# Autodesk Inventor assembly: Assembly
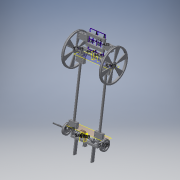
[picture p0: Inventor's stored thumbnail of the model, 180x180]
Saved by Autodesk Inventor 2018 (Build 220112000, 112)
## iProperties
Created: 2017-11-06
Part Number: Assembly
Document SubType Name: Assembly
Designer: David Cutting
Author: David Cutting
## Documents named in this file (17)
- C:\Users\Prakash\Documents\Inventor\MousetrapGit\Assembly.iam
- C:\Users\Prakash\Documents\Inventor\MousetrapGit\frontChassis_final.ipt
- C:\Users\Prakash\Documents\Inventor\MousetrapGit\carbonFiberTube.ipt
- C:\Users\Prakash\Documents\Inventor\MousetrapGit\clampCap.ipt
- C:\Users\Prakash\Documents\Inventor\MousetrapGit\rearChassis_final.ipt
- C:\Users\Prakash\Documents\Inventor\MousetrapGit\mousetrapHolder.ipt
- C:\Users\Prakash\Documents\Inventor\MousetrapGit\535018\bearings.ipt
- C:\Users\Prakash\Documents\Inventor\MousetrapGit\98873A200_MOISTURE-RESISTANT ACETAL THREADED ROD.ipt
- C:\Users\Prakash\Documents\Inventor\MousetrapGit\nutSecurer.ipt
- C:\Users\Prakash\Documents\Inventor\MousetrapGit\99223A029_ACETAL HEX NUT.ipt
- C:\Users\Prakash\Documents\Inventor\MousetrapGit\wheel.ipt
- C:\Users\Prakash\Documents\Inventor\MousetrapGit\spindleRod.ipt
- C:\Users\Prakash\Documents\Inventor\MousetrapGit\wheelSpindle.ipt
- C:\Users\Prakash\Documents\Inventor\MousetrapGit\intermediateSpindle.ipt
- C:\Users\Prakash\Documents\Inventor\MousetrapGit\wingnut_final.ipt
- C:\Users\Prakash\Documents\Inventor\MousetrapGit\washeript.ipt
- C:\Users\Prakash\Documents\Inventor\MousetrapGit\smallWheel.ipt
## Components (50 placed, 16 different names)
1. frontChassis_final:1 — Mate:1, Mate:2, Mate:3, Mate:4, Angle:3, Flush:3, Angle:4, Flush:4, Mate:16, Mate:17, Mate:18, Mate:19, Mate:24, Mate:25, Mate:26, Mate:27, Mate:52, Angle:8
2. carbonFiberTube:1 — Mate:1, Mate:2, Mate:6, Mate:9, Mate:10, Mate:12, Mate:14
3. carbonFiberTube:2 — Mate:3, Mate:4, Mate:5, Mate:7, Mate:8, Mate:11, Mate:13, Mate:15
4. clampCap:1 — Mate:8, Angle:1, Flush:1
5. clampCap:2 — Mate:9, Angle:2, Flush:2
6. rearChassis_final:1 — Mate:5, Mate:6, Mate:7, Angle:1, Flush:1, Angle:2, Flush:2, Mate:20, Mate:21, Mate:22, Mate:23, Mate:31, Angle:7
7. clampCap:3 — Mate:10, Angle:3, Flush:3
8. clampCap:4 — Mate:11, Angle:4, Flush:4
9. mousetrapHolder:1 — Mate:12, Mate:13, Angle:5, Flush:5, Angle:6, Flush:6
10. clampCap:5 — Mate:15, Angle:6, Flush:6
11. clampCap:6 — Mate:14, Angle:5, Flush:5
12. bearings:1 — Mate:16, Mate:17, Mate:29, Mate:35
13. bearings:2 — Mate:26, Mate:27
14. bearings:3 — Mate:18, Mate:19, Mate:28, Mate:39
15. bearings:4 — Mate:20, Mate:21, Mate:33
16. bearings:5 — Mate:24, Mate:25
17. bearings:6 — Mate:22, Mate:23, Mate:30, Mate:37
18. 98873A200_MOISTURE-RESISTANT ACETAL THREADED ROD:1 — Mate:30, Mate:31, Mate:32, Mate:36, Mate:40, Mate:42, Mate:49, Mate:50, Mate:62, Mate:64, Mate:65, Mate:76, Mate:79, Mate:80, Mate:82, Flush:7
19. 98873A200_MOISTURE-RESISTANT ACETAL THREADED ROD:2 — Mate:28, Mate:29, Mate:34, Mate:38, Mate:44, Mate:46, Mate:53, Mate:63, Mate:66, Mate:67, Mate:77, Mate:81, Mate:83, Mate:84, Flush:8, Mate:93, Mate:96
20. nutSecurer:1 — Mate:34, Mate:35, Mate:47
21. nutSecurer:2 — Mate:36, Mate:37, Mate:41
22. nutSecurer:3 — Mate:32, Mate:33, Mate:43
23. nutSecurer:4 — Mate:38, Mate:39, Mate:45
24. 99223A029_ACETAL HEX NUT:1 — Mate:40, Mate:41, Mate:68
25. 99223A029_ACETAL HEX NUT:2 — Mate:42, Mate:43, Mate:69
26. 99223A029_ACETAL HEX NUT:3 — Mate:46, Mate:47, Mate:70
27. 99223A029_ACETAL HEX NUT:4 — Mate:44, Mate:45, Mate:71
28. wheel:2 — Mate:50, Angle:11, Mate:74, Mate:87
29. wheel:4 — Mate:49, Angle:12, Mate:75, Mate:88
30. spindleRod:1 — Mate:52, Mate:54
31. wheelSpindle:1 — Mate:53, Flush:9
32. intermediateSpindle:1 — Mate:54, Flush:9
33. wingnut_final:1 — Mate:55, Mate:56, Mate:57, Mate:62, Angle:7
34. wingnut_final:2 — Mate:58, Mate:59, Mate:60, Mate:61, Mate:63, Angle:8
35. 99223A029_ACETAL HEX NUT:5 — Mate:55, Mate:56, Mate:57
36. 99223A029_ACETAL HEX NUT:6 — Mate:58, Mate:59, Mate:60, Mate:61
37. 99223A029_ACETAL HEX NUT:7 — Mate:64, Mate:68, Angle:12, Mate:75
38. 99223A029_ACETAL HEX NUT:8 — Mate:65, Mate:69, Angle:11, Mate:74
39. 99223A029_ACETAL HEX NUT:9 — Mate:67, Mate:71, Angle:14, Mate:97
40. 99223A029_ACETAL HEX NUT:10 — Mate:66, Mate:70, Angle:13, Mate:94
41. 99223A029_ACETAL HEX NUT:11 — Mate:77, Mate:91, Flush:8
42. 99223A029_ACETAL HEX NUT:12 — Mate:76, Mate:89
43. 99223A029_ACETAL HEX NUT:13 — Mate:79, Mate:90, Flush:7
44. washeript:1 — Mate:82, Mate:87, Mate:90
45. washeript:2 — Mate:81, Mate:91, Mate:98
46. washeript:4 — Mate:80, Mate:88, Mate:89
47. washeript:5 — Mate:83, Mate:92, Mate:95
48. 99223A029_ACETAL HEX NUT:14 — Mate:84, Mate:92
49. smallWheel:1 — Mate:93, Angle:13, Mate:94, Mate:95
50. smallWheel:2 — Mate:96, Angle:14, Mate:97, Mate:98
## Relationships (112: Mate 91, Angle 12, Flush 9)
- Mate:1: frontChassis_final:1 ↔ carbonFiberTube:1
- Mate:2: frontChassis_final:1 ↔ carbonFiberTube:1
- Mate:3: frontChassis_final:1 ↔ carbonFiberTube:2
- Mate:4: frontChassis_final:1 ↔ carbonFiberTube:2
- Mate:5: carbonFiberTube:2 ↔ rearChassis_final:1
- Mate:6: carbonFiberTube:1 ↔ rearChassis_final:1
- Mate:7: carbonFiberTube:2 ↔ rearChassis_final:1
- Mate:8: carbonFiberTube:2 ↔ clampCap:1
- Angle:1 (0 deg): clampCap:1 ↔ rearChassis_final:1
- Flush:1: clampCap:1 ↔ rearChassis_final:1
- Mate:9: carbonFiberTube:1 ↔ clampCap:2
- Angle:2 (0 deg): clampCap:2 ↔ rearChassis_final:1
- Flush:2: clampCap:2 ↔ rearChassis_final:1
- Mate:10: carbonFiberTube:1 ↔ clampCap:3
- Angle:3 (0 deg): frontChassis_final:1 ↔ clampCap:3
- Flush:3: frontChassis_final:1 ↔ clampCap:3
- Mate:11: carbonFiberTube:2 ↔ clampCap:4
- Angle:4 (0 deg): frontChassis_final:1 ↔ clampCap:4
- Flush:4: frontChassis_final:1 ↔ clampCap:4
- Mate:12: carbonFiberTube:1 ↔ mousetrapHolder:1
- Mate:13: carbonFiberTube:2 ↔ mousetrapHolder:1
- Mate:14: carbonFiberTube:1 ↔ clampCap:6
- Angle:5 (0 deg): mousetrapHolder:1 ↔ clampCap:6
- Flush:5: mousetrapHolder:1 ↔ clampCap:6
- Mate:15: carbonFiberTube:2 ↔ clampCap:5
- Angle:6 (0 deg): mousetrapHolder:1 ↔ clampCap:5
- Flush:6: mousetrapHolder:1 ↔ clampCap:5
- Mate:16: frontChassis_final:1 ↔ bearings:1
- Mate:17: frontChassis_final:1 ↔ bearings:1
- Mate:18: frontChassis_final:1 ↔ bearings:3
- Mate:19: frontChassis_final:1 ↔ bearings:3
- Mate:20: rearChassis_final:1 ↔ bearings:4
- Mate:21: rearChassis_final:1 ↔ bearings:4
- Mate:22: rearChassis_final:1 ↔ bearings:6
- Mate:23: rearChassis_final:1 ↔ bearings:6
- Mate:24: frontChassis_final:1 ↔ bearings:5
- Mate:25: frontChassis_final:1 ↔ bearings:5
- Mate:26: frontChassis_final:1 ↔ bearings:2
- Mate:27: frontChassis_final:1 ↔ bearings:2
- Mate:28: bearings:3 ↔ 98873A200_MOISTURE-RESISTANT ACETAL THREADED ROD:2
- Mate:29: bearings:1 ↔ 98873A200_MOISTURE-RESISTANT ACETAL THREADED ROD:2
- Mate:30: bearings:6 ↔ 98873A200_MOISTURE-RESISTANT ACETAL THREADED ROD:1
- Mate:31: rearChassis_final:1 ↔ 98873A200_MOISTURE-RESISTANT ACETAL THREADED ROD:1
- Mate:32: 98873A200_MOISTURE-RESISTANT ACETAL THREADED ROD:1 ↔ nutSecurer:3
- Mate:33: bearings:4 ↔ nutSecurer:3
- Mate:34: 98873A200_MOISTURE-RESISTANT ACETAL THREADED ROD:2 ↔ nutSecurer:1
- Mate:35: bearings:1 ↔ nutSecurer:1
- Mate:36: 98873A200_MOISTURE-RESISTANT ACETAL THREADED ROD:1 ↔ nutSecurer:2
- Mate:37: bearings:6 ↔ nutSecurer:2
- Mate:38: 98873A200_MOISTURE-RESISTANT ACETAL THREADED ROD:2 ↔ nutSecurer:4
- Mate:39: bearings:3 ↔ nutSecurer:4
- Mate:40: 98873A200_MOISTURE-RESISTANT ACETAL THREADED ROD:1 ↔ 99223A029_ACETAL HEX NUT:1
- Mate:41: nutSecurer:2 ↔ 99223A029_ACETAL HEX NUT:1
- Mate:42: 98873A200_MOISTURE-RESISTANT ACETAL THREADED ROD:1 ↔ 99223A029_ACETAL HEX NUT:2
- Mate:43: nutSecurer:3 ↔ 99223A029_ACETAL HEX NUT:2
- Mate:44: 98873A200_MOISTURE-RESISTANT ACETAL THREADED ROD:2 ↔ 99223A029_ACETAL HEX NUT:4
- Mate:45: nutSecurer:4 ↔ 99223A029_ACETAL HEX NUT:4
- Mate:46: 98873A200_MOISTURE-RESISTANT ACETAL THREADED ROD:2 ↔ 99223A029_ACETAL HEX NUT:3
- Mate:47: nutSecurer:1 ↔ 99223A029_ACETAL HEX NUT:3
- Mate:49: 98873A200_MOISTURE-RESISTANT ACETAL THREADED ROD:1 ↔ wheel:4
- Mate:50: 98873A200_MOISTURE-RESISTANT ACETAL THREADED ROD:1 ↔ wheel:2
- Mate:52: frontChassis_final:1 ↔ spindleRod:1
- Mate:53: 98873A200_MOISTURE-RESISTANT ACETAL THREADED ROD:2 ↔ wheelSpindle:1
- Mate:54: spindleRod:1 ↔ intermediateSpindle:1
- Mate:55: wingnut_final:1 ↔ 99223A029_ACETAL HEX NUT:5
- Mate:56: wingnut_final:1 ↔ 99223A029_ACETAL HEX NUT:5
- Mate:57: wingnut_final:1 ↔ 99223A029_ACETAL HEX NUT:5
- Mate:58: wingnut_final:2 ↔ 99223A029_ACETAL HEX NUT:6
- Mate:59: wingnut_final:2 ↔ 99223A029_ACETAL HEX NUT:6
- Mate:60: wingnut_final:2 ↔ 99223A029_ACETAL HEX NUT:6
- Mate:61: wingnut_final:2 ↔ 99223A029_ACETAL HEX NUT:6
- Mate:62: 98873A200_MOISTURE-RESISTANT ACETAL THREADED ROD:1 ↔ wingnut_final:1
- Angle:7 (0 deg): rearChassis_final:1 ↔ wingnut_final:1
- Mate:63: 98873A200_MOISTURE-RESISTANT ACETAL THREADED ROD:2 ↔ wingnut_final:2
- Angle:8 (0 deg): frontChassis_final:1 ↔ wingnut_final:2
- Mate:64: 98873A200_MOISTURE-RESISTANT ACETAL THREADED ROD:1 ↔ 99223A029_ACETAL HEX NUT:7
- Mate:65: 98873A200_MOISTURE-RESISTANT ACETAL THREADED ROD:1 ↔ 99223A029_ACETAL HEX NUT:8
- Mate:66: 98873A200_MOISTURE-RESISTANT ACETAL THREADED ROD:2 ↔ 99223A029_ACETAL HEX NUT:10
- Mate:67: 98873A200_MOISTURE-RESISTANT ACETAL THREADED ROD:2 ↔ 99223A029_ACETAL HEX NUT:9
- Mate:68: 99223A029_ACETAL HEX NUT:1 ↔ 99223A029_ACETAL HEX NUT:7
- Mate:69: 99223A029_ACETAL HEX NUT:2 ↔ 99223A029_ACETAL HEX NUT:8
- Mate:70: 99223A029_ACETAL HEX NUT:3 ↔ 99223A029_ACETAL HEX NUT:10
- Mate:71: 99223A029_ACETAL HEX NUT:4 ↔ 99223A029_ACETAL HEX NUT:9
- Angle:11 (0 deg): wheel:2 ↔ 99223A029_ACETAL HEX NUT:8
- Mate:74: wheel:2 ↔ 99223A029_ACETAL HEX NUT:8
- Angle:12 (0 deg): wheel:4 ↔ 99223A029_ACETAL HEX NUT:7
- Mate:75: wheel:4 ↔ 99223A029_ACETAL HEX NUT:7
- Mate:76: 98873A200_MOISTURE-RESISTANT ACETAL THREADED ROD:1 ↔ 99223A029_ACETAL HEX NUT:12
- Mate:77: 98873A200_MOISTURE-RESISTANT ACETAL THREADED ROD:2 ↔ 99223A029_ACETAL HEX NUT:11
- Mate:79: 98873A200_MOISTURE-RESISTANT ACETAL THREADED ROD:1 ↔ 99223A029_ACETAL HEX NUT:13
- Mate:80: 98873A200_MOISTURE-RESISTANT ACETAL THREADED ROD:1 ↔ washeript:4
- Mate:81: 98873A200_MOISTURE-RESISTANT ACETAL THREADED ROD:2 ↔ washeript:2
- Mate:82: 98873A200_MOISTURE-RESISTANT ACETAL THREADED ROD:1 ↔ washeript:1
- Mate:83: 98873A200_MOISTURE-RESISTANT ACETAL THREADED ROD:2 ↔ washeript:5
- Mate:84: 98873A200_MOISTURE-RESISTANT ACETAL THREADED ROD:2 ↔ 99223A029_ACETAL HEX NUT:14
- Mate:87: wheel:2 ↔ washeript:1
- Mate:88: wheel:4 ↔ washeript:4
- Mate:89: 99223A029_ACETAL HEX NUT:12 ↔ washeript:4
- Mate:90: 99223A029_ACETAL HEX NUT:13 ↔ washeript:1
- Mate:91: 99223A029_ACETAL HEX NUT:11 ↔ washeript:2
- Mate:92: washeript:5 ↔ 99223A029_ACETAL HEX NUT:14
- Flush:7: 98873A200_MOISTURE-RESISTANT ACETAL THREADED ROD:1 ↔ 99223A029_ACETAL HEX NUT:13
- Flush:8: 98873A200_MOISTURE-RESISTANT ACETAL THREADED ROD:2 ↔ 99223A029_ACETAL HEX NUT:11
- Flush:9: wheelSpindle:1 ↔ intermediateSpindle:1
- Mate:93: 98873A200_MOISTURE-RESISTANT ACETAL THREADED ROD:2 ↔ smallWheel:1
- Angle:13 (0 deg): 99223A029_ACETAL HEX NUT:10 ↔ smallWheel:1
- Mate:94: 99223A029_ACETAL HEX NUT:10 ↔ smallWheel:1
- Mate:95: washeript:5 ↔ smallWheel:1
- Mate:96: 98873A200_MOISTURE-RESISTANT ACETAL THREADED ROD:2 ↔ smallWheel:2
- Angle:14 (0 deg): 99223A029_ACETAL HEX NUT:9 ↔ smallWheel:2
- Mate:97: 99223A029_ACETAL HEX NUT:9 ↔ smallWheel:2
- Mate:98: washeript:2 ↔ smallWheel:2
